# Autodesk Inventor assembly: 組合2
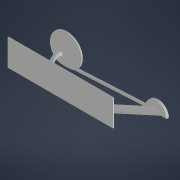
[picture p0: Inventor's stored thumbnail of the model, 180x180]
Saved by Autodesk Inventor 2021 (Build 250183000, 183)
## iProperties
Created: 2021-01-06
Part Number: 組合2
Document SubType Name: Assembly
Designer: zihon
Author: zihon
## Documents named in this file (8)
- C:\Users\zihon\Desktop\New folder\組合2.iam
- C:\Users\zihon\Desktop\New folder\架2.ipt
- C:\Users\zihon\Desktop\New folder\螺旋2.ipt
- C:\Users\zihon\Desktop\New folder\零件1.ipt
- C:\Users\zihon\Desktop\New folder\零件2.ipt
- C:\Users\zihon\Desktop\New folder\零件3.ipt
- C:\Users\zihon\Desktop\New folder\零件4.ipt
- C:\Users\zihon\Desktop\New folder\軸.ipt
## Components (7 placed, 7 different names)
1. 架2:1 — 齊平:1, 貼合:1, 齊平:2, 貼合:2, 貼合:3, 貼合:4, 貼合:5, 貼合:12, 貼合:13, 貼合:14, 貼合:15, 貼合:16, 貼合:17, 貼合:18, 貼合:19
2. 螺旋2:1 — 貼合:2, 貼合:3
3. 零件1:1 — 貼合:4, 貼合:5, 相切:1
4. 零件2:1 — 貼合:14, 貼合:15, 相切:5
5. 零件3:1 — 貼合:16, 貼合:17, 相切:6
6. 零件4:1 — 貼合:18, 貼合:19, 相切:7
7. 軸:1 — 貼合:12, 貼合:13, 相切:1, 相切:5, 相切:6, 相切:7
## Relationships (19: Mate 13, Tangent 4, Flush 2)
- 齊平:1 [Flush]: 架2:1
- 貼合:1 [Mate]: 架2:1
- 齊平:2 [Flush]: 架2:1
- 貼合:2 [Mate]: 架2:1 ↔ 螺旋2:1
- 貼合:3 [Mate]: 架2:1 ↔ 螺旋2:1
- 貼合:4 [Mate]: 架2:1 ↔ 零件1:1
- 貼合:5 [Mate]: 架2:1 ↔ 零件1:1
- 貼合:12 [Mate]: 架2:1 ↔ 軸:1
- 貼合:13 [Mate]: 架2:1 ↔ 軸:1
- 相切:1 [Tangent]: 零件1:1 ↔ 軸:1
- 貼合:14 [Mate]: 架2:1 ↔ 零件2:1
- 貼合:15 [Mate]: 架2:1 ↔ 零件2:1
- 相切:5 [Tangent]: 零件2:1 ↔ 軸:1
- 貼合:16 [Mate]: 架2:1 ↔ 零件3:1
- 貼合:17 [Mate]: 架2:1 ↔ 零件3:1
- 相切:6 [Tangent]: 零件3:1 ↔ 軸:1
- 貼合:18 [Mate]: 架2:1 ↔ 零件4:1
- 貼合:19 [Mate]: 架2:1 ↔ 零件4:1
- 相切:7 [Tangent]: 零件4:1 ↔ 軸:1
